# Autodesk Inventor assembly: VER2.0_MIR
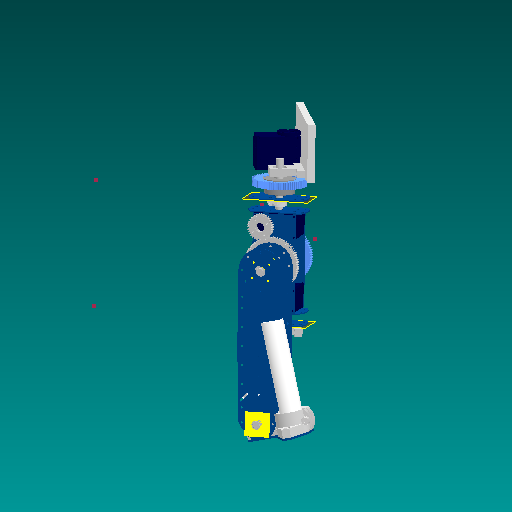
[picture p0: Inventor's stored thumbnail of the model, 512x512]
Saved by Autodesk Inventor 2020 (Build 240168000, 168)
## iProperties
Created: 2022-10-31
Part Number: VER2.0_MIR
Document SubType Name: Assembly
Designer: kanazawakotaro
Author: Administrator
## Documents named in this file (25)
- C:\Users\金澤航太郎\Documents\Inventor\kamuy2\VER2.0_MIR.iam
- C:\Users\金澤航太郎\Documents\Inventor\kamuy2\Parts\Part2_MIR.ipt
- C:\Users\金澤航太郎\Documents\Inventor\kamuy2\Parts\x-540_idle_MIR.ipt
- C:\Users\金澤航太郎\Documents\Inventor\kamuy2\Parts\GEABP1.0-32-10-A-12-KFC22-K3_Autodesk_Inventor_2020_20221101\AIS2020\GEABP1_0-32-10-A-12-KFC22-K3_MIR.iam
- C:\Users\金澤航太郎\Documents\Inventor\kamuy2\Parts\GEYK1.0-70-10-B-10K_Autodesk_Inventor_2020_20221114\AIS2020\GEYK1_0-70-10-B-10K_MIR.iam
- C:\Users\金澤航太郎\Documents\Inventor\kamuy2\Parts\GEABP1.0-70-10-A-19-KFC30-K3_Autodesk_Inventor_2020_20221114\AIS2020\GEABP1_0-70-10-A-19-KFC30-K3_MIR.iam
- C:\Users\金澤航太郎\Documents\Inventor\kamuy2\Parts\PIJX30-20-150_Autodesk_Inventor_2020_20221115\PIJX30-20-150_MIR.ipt
- C:\Users\金澤航太郎\Documents\Inventor\kamuy2\Parts\C-SHA10_Autodesk_Inventor_2020_20221104\AIS2020\C-SHA10_MIR.iam
- C:\Users\金澤航太郎\Documents\Inventor\kamuy2\Part16_MIR.ipt
- C:\Users\金澤航太郎\Documents\Inventor\kamuy2\Parts\HTPA30S3M060-A-N10_Autodesk_Inventor_2020_20221115\AIS2020\HTPA30S3M060-A-N10_MIR.iam
- C:\Users\金澤航太郎\Documents\Inventor\kamuy2\Part1_MIR.ipt
- C:\Users\金澤航太郎\Documents\Inventor\kamuy2\Part13_MIR.ipt
- C:\Users\金澤航太郎\Documents\Inventor\kamuy2\Part17_MIR.ipt
- C:\Users\金澤航太郎\Documents\Inventor\kamuy2\Parts\SMYHF10_STEP_AP203AP214\SMYHF10_203_MIR.ipt
- C:\Users\金澤航太郎\Documents\Inventor\kamuy2\Part19_MIR.ipt
- C:\Users\金澤航太郎\Documents\Inventor\kamuy2\Parts\BGHK6800VV-30_Autodesk_Inventor_2020_20221102\AIS2020\BGHK6800VV-30_MIR.iam
- C:\Users\金澤航太郎\Documents\Inventor\kamuy2\Parts\XW540.N105.I101_MIR.ipt
- C:\Users\金澤航太郎\Documents\Inventor\kamuy2\Parts\NSFMKR10-67-KA22-A20_Autodesk_Inventor_2020_20221116\AIS2020\NSFMKR10-67-KA22-A20_MIR.iam
- C:\Users\金澤航太郎\Documents\Inventor\kamuy2\Parts\NSFMR10-37_Autodesk_Inventor_2020_20221116\AIS2020\NSFMR10-37(000_000)_MIR.iam
- C:\Users\金澤航太郎\Documents\Inventor\kamuy2\Part20_MIR.ipt
- C:\Users\金澤航太郎\Documents\Inventor\kamuy2\Parts\SMYHF30_STEP_AP203AP214\SMYHF30_203_MIR.ipt
- C:\Users\金澤航太郎\Documents\Inventor\kamuy2\Part22_MIR.ipt
- C:\Users\金澤航太郎\Documents\Inventor\kamuy2\Parts\RORPOS20-L30_Autodesk_Inventor_2020_20221117\AIS2020\RORPOS20-L30_MIR.iam
- C:\Users\金澤航太郎\Documents\Inventor\kamuy2\Parts\NSFMRRA10-74-B3-S3-KC31.5-A11_Autodesk_Inventor_2020_20221116\AIS2020\NSFMRRA10-74-B3-S3-KC31_5-A11(000_000)_MIR.iam
- C:\Users\金澤航太郎\Documents\Inventor\kamuy2\Parts\NSFMKRRA10-144-F3-S6-KA5-A18-KB108.5-B11_Autodesk_Inventor_2020_20221117\AIS2020\NSFMKRRA10-144-F3-S6-KA5-A18-KB108_5-B11_MIR.iam
## Components (40 placed, 24 different names)
1. Part2_MIR:1
2. x-540_idle_MIR:1 — メイト:51, メイト:50, フラッシュ:68, フラッシュ:66, フラッシュ:58, メイト:258, メイト:154, フラッシュ:140, メイト:166, フラッシュ:103, メイト:256
3. GEABP1_0-32-10-A-12-KFC22-K3_MIR:1 [sub-assembly] — メイト:51, メイト:50, フラッシュ:69
4. GEYK1_0-70-10-B-10K_MIR:1 [sub-assembly] — フラッシュ:61, フラッシュ:136, メイト:248
5. x-540_idle_MIR:2 — フラッシュ:68, フラッシュ:66, フラッシュ:58, メイト:86, メイト:85, メイト:168, フラッシュ:100, メイト:183, メイト:180, メイト:179, メイト:178
6. GEABP1_0-32-10-A-12-KFC22-K3_MIR:2 [sub-assembly] — フラッシュ:61, メイト:86, メイト:85
7. GEABP1_0-70-10-A-19-KFC30-K3_MIR:1 [sub-assembly] — フラッシュ:69, フラッシュ:123, メイト:255
8. PIJX30-20-150_MIR:1 — メイト:244, メイト:245
9. C-SHA10_MIR:1 [sub-assembly] — フラッシュ:131, フラッシュ:89, メイト:235, メイト:249, フラッシュ:133, メイト:264
10. C-SHA10_MIR:2 [sub-assembly] — フラッシュ:131, フラッシュ:89, メイト:237, メイト:250
11. Part16_MIR:1 — フラッシュ:96, フラッシュ:122, メイト:236
12. Part16_MIR:2 — メイト:258, フラッシュ:92, メイト:170
13. Part16_MIR:3 — メイト:168, メイト:154, フラッシュ:92, フラッシュ:121, フラッシュ:93, フラッシュ:141, メイト:171
14. Part16_MIR:4 — フラッシュ:121, フラッシュ:96, フラッシュ:93, メイト:219, メイト:164, メイト:230
15. Part16_MIR:5 — フラッシュ:122, メイト:219, メイト:234, フラッシュ:139, メイト:252
16. HTPA30S3M060-A-N10_MIR:1 [sub-assembly] — フラッシュ:138, メイト:263
17. HTPA30S3M060-A-N10_MIR:2 [sub-assembly] — フラッシュ:138, メイト:164, メイト:259
18. Part1_MIR:1 — フラッシュ:141, フラッシュ:140, メイト:171, フラッシュ:100, フラッシュ:101
19. Part1_MIR:2 — メイト:183, メイト:170, メイト:166, フラッシュ:101, メイト:257
20. Part13_MIR:1 — フラッシュ:103, フラッシュ:108, フラッシュ:104, メイト:172, メイト:208
21. Part17_MIR:1 — フラッシュ:108, フラッシュ:104, メイト:172, フラッシュ:105, メイト:174, メイト:177
22. SMYHF10_203_MIR:1 — フラッシュ:105, メイト:174, メイト:254
23. GEYK1_0-70-10-B-10K_MIR:2 [sub-assembly] — メイト:177, メイト:200, メイト:207
24. Part13_MIR:2 — メイト:180, メイト:179, メイト:178, フラッシュ:110, メイト:194, メイト:214
25. SMYHF10_203_MIR:2 — メイト:187, メイト:185, メイト:213
26. Part17_MIR:2 — フラッシュ:110, メイト:194, メイト:187, メイト:185, メイト:211, メイト:215
27. Part19_MIR:1 — メイト:200, メイト:206, フラッシュ:113, フラッシュ:114, メイト:202
28. BGHK6800VV-30_MIR:1 [sub-assembly] — メイト:206, フラッシュ:113, メイト:205, メイト:209, フラッシュ:116, フラッシュ:115
29. GEABP1_0-32-10-A-12-KFC22-K3_MIR:3 [sub-assembly] — メイト:204, メイト:203
30. XW540.N105.I101_MIR:1 — メイト:205, メイト:204, メイト:203, フラッシュ:114, メイト:202
31. NSFMKR10-67-KA22-A20_MIR:1 [sub-assembly] — メイト:254, メイト:209, メイト:208, メイト:207
32. BGHK6800VV-30_MIR:2 [sub-assembly] — メイト:211, フラッシュ:116, フラッシュ:115, メイト:212
33. NSFMR10-37(000_000)_MIR:1 [sub-assembly] — メイト:215, メイト:214, メイト:213, メイト:212
34. Part20_MIR:1 — メイト:237, メイト:236, フラッシュ:123, メイト:265, フラッシュ:142, メイト:261
35. Part20_MIR:2 — メイト:265, フラッシュ:142, メイト:235, メイト:234, メイト:230, メイト:251, メイト:247, メイト:253, フラッシュ:137
36. SMYHF30_203_MIR:1 — メイト:244, メイト:246, フラッシュ:135, メイト:242
37. Part22_MIR:1 — メイト:250, メイト:249, メイト:246, フラッシュ:135, メイト:245, メイト:242, フラッシュ:133
38. RORPOS20-L30_MIR:1 [sub-assembly] — メイト:251, メイト:247
39. NSFMRRA10-74-B3-S3-KC31_5-A11(000_000)_MIR:1 [sub-assembly] — メイト:264, メイト:263, メイト:253, フラッシュ:139, メイト:252
40. NSFMKRRA10-144-F3-S6-KA5-A18-KB108_5-B11_MIR:1 [sub-assembly] — メイト:261, メイト:259, メイト:257, メイト:256, メイト:255, フラッシュ:137, フラッシュ:136, メイト:248
## Relationships (94: Mate 65, Flush 29)
- メイト:51 [Mate]: x-540_idle_MIR:1 ↔ GEABP1_0-32-10-A-12-KFC22-K3_MIR:1
- メイト:50 [Mate] (4 mm): x-540_idle_MIR:1 ↔ GEABP1_0-32-10-A-12-KFC22-K3_MIR:1
- フラッシュ:68 [Flush]: x-540_idle_MIR:1 ↔ x-540_idle_MIR:2
- フラッシュ:66 [Flush]: x-540_idle_MIR:1 ↔ x-540_idle_MIR:2
- フラッシュ:58 [Flush]: x-540_idle_MIR:1 ↔ x-540_idle_MIR:2
- フラッシュ:61 [Flush]: GEYK1_0-70-10-B-10K_MIR:1 ↔ GEABP1_0-32-10-A-12-KFC22-K3_MIR:2
- メイト:86 [Mate] (4 mm): x-540_idle_MIR:2 ↔ GEABP1_0-32-10-A-12-KFC22-K3_MIR:2
- メイト:85 [Mate]: x-540_idle_MIR:2 ↔ GEABP1_0-32-10-A-12-KFC22-K3_MIR:2
- フラッシュ:69 [Flush]: GEABP1_0-32-10-A-12-KFC22-K3_MIR:1 ↔ GEABP1_0-70-10-A-19-KFC30-K3_MIR:1
- フラッシュ:131 [Flush]: C-SHA10_MIR:1 ↔ C-SHA10_MIR:2
- フラッシュ:89 [Flush]: C-SHA10_MIR:1 ↔ C-SHA10_MIR:2
- メイト:258 [Mate] (15.591 mm): x-540_idle_MIR:1 ↔ Part16_MIR:2
- メイト:168 [Mate] (15.591 mm): x-540_idle_MIR:2 ↔ Part16_MIR:3
- メイト:154 [Mate] (15.591 mm): x-540_idle_MIR:1 ↔ Part16_MIR:3
- フラッシュ:92 [Flush]: Part16_MIR:2 ↔ Part16_MIR:3
- フラッシュ:121 [Flush]: Part16_MIR:3 ↔ Part16_MIR:4
- フラッシュ:96 [Flush]: Part16_MIR:1 ↔ Part16_MIR:4
- フラッシュ:93 [Flush]: Part16_MIR:3 ↔ Part16_MIR:4
- フラッシュ:122 [Flush]: Part16_MIR:1 ↔ Part16_MIR:5
- メイト:219 [Mate] (168 mm): Part16_MIR:4 ↔ Part16_MIR:5
- フラッシュ:138 [Flush]: HTPA30S3M060-A-N10_MIR:1 ↔ HTPA30S3M060-A-N10_MIR:2
- メイト:164 [Mate] (7 mm): Part16_MIR:4 ↔ HTPA30S3M060-A-N10_MIR:2
- フラッシュ:141 [Flush] (12.859 mm): Part16_MIR:3 ↔ Part1_MIR:1
- フラッシュ:140 [Flush]: x-540_idle_MIR:1 ↔ Part1_MIR:1
- メイト:171 [Mate]: Part16_MIR:3 ↔ Part1_MIR:1
- フラッシュ:100 [Mate]: x-540_idle_MIR:2 ↔ Part1_MIR:1
- メイト:183 [Mate]: x-540_idle_MIR:2 ↔ Part1_MIR:2
- メイト:170 [Mate]: Part16_MIR:2 ↔ Part1_MIR:2
- メイト:166 [Mate]: x-540_idle_MIR:1 ↔ Part1_MIR:2
- フラッシュ:101 [Flush]: Part1_MIR:1 ↔ Part1_MIR:2
- フラッシュ:103 [Mate]: x-540_idle_MIR:1 ↔ Part13_MIR:1
- フラッシュ:108 [Flush]: Part13_MIR:1 ↔ Part17_MIR:1
- フラッシュ:104 [Flush]: Part13_MIR:1 ↔ Part17_MIR:1
- メイト:172 [Mate] (15 mm): Part13_MIR:1 ↔ Part17_MIR:1
- フラッシュ:105 [Flush] (0.1 mm): Part17_MIR:1 ↔ SMYHF10_203_MIR:1
- メイト:174 [Mate]: Part17_MIR:1 ↔ SMYHF10_203_MIR:1
- メイト:177 [Mate] (5 mm): Part17_MIR:1 ↔ GEYK1_0-70-10-B-10K_MIR:2
- メイト:180 [Mate]: x-540_idle_MIR:2 ↔ Part13_MIR:2
- メイト:179 [Mate]: x-540_idle_MIR:2 ↔ Part13_MIR:2
- メイト:178 [Mate]: x-540_idle_MIR:2 ↔ Part13_MIR:2
- フラッシュ:110 [Flush]: Part13_MIR:2 ↔ Part17_MIR:2
- メイト:194 [Mate] (15 mm): Part13_MIR:2 ↔ Part17_MIR:2
- メイト:187 [Mate]: SMYHF10_203_MIR:2 ↔ Part17_MIR:2
- メイト:185 [Mate]: SMYHF10_203_MIR:2 ↔ Part17_MIR:2
- メイト:200 [Mate] (4 mm): GEYK1_0-70-10-B-10K_MIR:2 ↔ Part19_MIR:1
- メイト:206 [Mate]: Part19_MIR:1 ↔ BGHK6800VV-30_MIR:1
- フラッシュ:113 [Flush]: Part19_MIR:1 ↔ BGHK6800VV-30_MIR:1
- メイト:205 [Mate] (6.591 mm): BGHK6800VV-30_MIR:1 ↔ XW540.N105.I101_MIR:1
- メイト:204 [Mate]: GEABP1_0-32-10-A-12-KFC22-K3_MIR:3 ↔ XW540.N105.I101_MIR:1
- メイト:203 [Mate]: GEABP1_0-32-10-A-12-KFC22-K3_MIR:3 ↔ XW540.N105.I101_MIR:1
- フラッシュ:114 [Flush]: Part19_MIR:1 ↔ XW540.N105.I101_MIR:1
- メイト:202 [Mate]: Part19_MIR:1 ↔ XW540.N105.I101_MIR:1
- メイト:254 [Mate]: SMYHF10_203_MIR:1 ↔ NSFMKR10-67-KA22-A20_MIR:1
- メイト:209 [Mate]: BGHK6800VV-30_MIR:1 ↔ NSFMKR10-67-KA22-A20_MIR:1
- メイト:208 [Mate]: Part13_MIR:1 ↔ NSFMKR10-67-KA22-A20_MIR:1
- メイト:207 [Mate]: GEYK1_0-70-10-B-10K_MIR:2 ↔ NSFMKR10-67-KA22-A20_MIR:1
- メイト:211 [Mate] (4 mm): Part17_MIR:2 ↔ BGHK6800VV-30_MIR:2
- フラッシュ:116 [Flush]: BGHK6800VV-30_MIR:1 ↔ BGHK6800VV-30_MIR:2
- フラッシュ:115 [Flush]: BGHK6800VV-30_MIR:1 ↔ BGHK6800VV-30_MIR:2
- メイト:215 [Mate]: Part17_MIR:2 ↔ NSFMR10-37(000_000)_MIR:1
- メイト:214 [Mate]: Part13_MIR:2 ↔ NSFMR10-37(000_000)_MIR:1
- メイト:213 [Mate]: SMYHF10_203_MIR:2 ↔ NSFMR10-37(000_000)_MIR:1
- メイト:212 [Mate]: BGHK6800VV-30_MIR:2 ↔ NSFMR10-37(000_000)_MIR:1
- メイト:237 [Mate] (6 mm): C-SHA10_MIR:2 ↔ Part20_MIR:1
- メイト:236 [Mate]: Part16_MIR:1 ↔ Part20_MIR:1
- フラッシュ:123 [Mate]: GEABP1_0-70-10-A-19-KFC30-K3_MIR:1 ↔ Part20_MIR:1
- メイト:265 [Mate]: Part20_MIR:1 ↔ Part20_MIR:2
- フラッシュ:142 [Flush]: Part20_MIR:1 ↔ Part20_MIR:2
- メイト:235 [Mate] (6 mm): C-SHA10_MIR:1 ↔ Part20_MIR:2
- メイト:234 [Mate]: Part16_MIR:5 ↔ Part20_MIR:2
- メイト:230 [Mate]: Part16_MIR:4 ↔ Part20_MIR:2
- メイト:244 [Mate]: PIJX30-20-150_MIR:1 ↔ SMYHF30_203_MIR:1
- メイト:250 [Mate]: C-SHA10_MIR:2 ↔ Part22_MIR:1
- メイト:249 [Mate]: C-SHA10_MIR:1 ↔ Part22_MIR:1
- メイト:246 [Mate]: SMYHF30_203_MIR:1 ↔ Part22_MIR:1
- フラッシュ:135 [Flush]: SMYHF30_203_MIR:1 ↔ Part22_MIR:1
- メイト:245 [Mate]: PIJX30-20-150_MIR:1 ↔ Part22_MIR:1
- メイト:242 [Mate]: SMYHF30_203_MIR:1 ↔ Part22_MIR:1
- フラッシュ:133 [Mate]: C-SHA10_MIR:1 ↔ Part22_MIR:1
- メイト:251 [Mate]: Part20_MIR:2 ↔ RORPOS20-L30_MIR:1
- メイト:247 [Mate] (2.5 mm): Part20_MIR:2 ↔ RORPOS20-L30_MIR:1
- メイト:264 [Mate]: C-SHA10_MIR:1 ↔ NSFMRRA10-74-B3-S3-KC31_5-A11(000_000)_MIR:1
- メイト:263 [Mate]: HTPA30S3M060-A-N10_MIR:1 ↔ NSFMRRA10-74-B3-S3-KC31_5-A11(000_000)_MIR:1
- メイト:253 [Mate]: Part20_MIR:2 ↔ NSFMRRA10-74-B3-S3-KC31_5-A11(000_000)_MIR:1
- フラッシュ:139 [Flush] (-3 mm): Part16_MIR:5 ↔ NSFMRRA10-74-B3-S3-KC31_5-A11(000_000)_MIR:1
- メイト:252 [Mate]: Part16_MIR:5 ↔ NSFMRRA10-74-B3-S3-KC31_5-A11(000_000)_MIR:1
- メイト:261 [Mate]: Part20_MIR:1 ↔ NSFMKRRA10-144-F3-S6-KA5-A18-KB108_5-B11_MIR:1
- メイト:259 [Mate]: HTPA30S3M060-A-N10_MIR:2 ↔ NSFMKRRA10-144-F3-S6-KA5-A18-KB108_5-B11_MIR:1
- メイト:257 [Mate] (-28.819 mm): Part1_MIR:2 ↔ NSFMKRRA10-144-F3-S6-KA5-A18-KB108_5-B11_MIR:1
- メイト:256 [Mate] (31.591 mm): x-540_idle_MIR:1 ↔ NSFMKRRA10-144-F3-S6-KA5-A18-KB108_5-B11_MIR:1
- メイト:255 [Mate]: GEABP1_0-70-10-A-19-KFC30-K3_MIR:1 ↔ NSFMKRRA10-144-F3-S6-KA5-A18-KB108_5-B11_MIR:1
- フラッシュ:137 [Flush] (6 mm): Part20_MIR:2 ↔ NSFMKRRA10-144-F3-S6-KA5-A18-KB108_5-B11_MIR:1
- フラッシュ:136 [Flush] (-3 mm): GEYK1_0-70-10-B-10K_MIR:1 ↔ NSFMKRRA10-144-F3-S6-KA5-A18-KB108_5-B11_MIR:1
- メイト:248 [Mate]: GEYK1_0-70-10-B-10K_MIR:1 ↔ NSFMKRRA10-144-F3-S6-KA5-A18-KB108_5-B11_MIR:1
